# Autodesk Inventor assembly: Shoulder V2
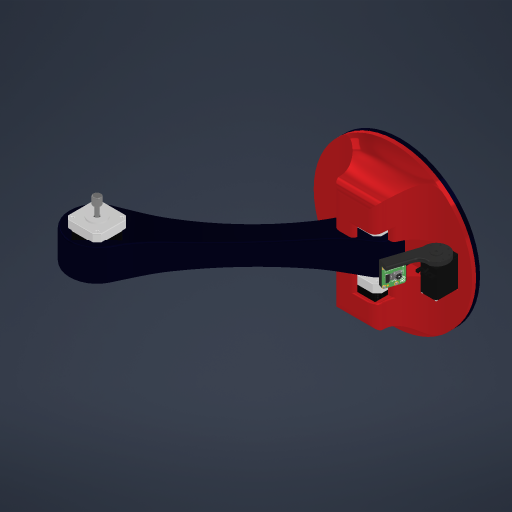
[picture p0: Inventor's stored thumbnail of the model, 512x512]
Saved by Autodesk Inventor 2023 (Build 270158000, 158)
## iProperties
Created: 2023-04-08
Part Number: Shoulder V2
Document SubType Name: Assembly
Designer: vatdu
Author: vatdu
## Documents named in this file (8)
- C:\Users\vatdu\Desktop\CRYSTAL MARK II\Arm\Shoulder\Shoulder V2.iam
- C:\Users\vatdu\Desktop\CRYSTAL MARK II\Components\Stepper Motor.ipt
- C:\Users\vatdu\Desktop\CRYSTAL MARK II\Arm\Shoulder\Rotating Plate.ipt
- C:\Users\vatdu\Desktop\CRYSTAL MARK II\Arm\Shoulder\Motor Cover V2.ipt
- C:\Users\vatdu\Desktop\CRYSTAL MARK II\Arm\Shoulder\Arm.ipt
- C:\Users\vatdu\Desktop\CRYSTAL MARK II\Components\Servo.ipt
- C:\Users\vatdu\Desktop\CRYSTAL MARK II\Components\Camera.iam
- C:\Users\vatdu\Documents\Inventor\Content Center Files\R2023\en-US\BS EN ISO 7045 H\EN ISO 7045 - M1.6 x 3 - 4.8 - H(1).ipt
## Components (13 placed, 7 different names)
1. Stepper Motor:1 — Rigid:3
2. Stepper Motor:2 — Rigid:4, Rigid:6
3. Stepper Motor:3 — Rigid:1, Rotational:2, Rigid:5
4. Rotating Plate:1 — Rotational:1
5. Motor Cover V2:1 — Rigid:1, Rigid:3, Rotational:1
6. Arm:1 — Rigid:4, Rotational:2, Rigid:5, Rigid:6
7. Servo:1 — Rotational:3
8. Camera:1 [sub-assembly] — Rotational:3, Insert:1, Insert:2, Insert:3, Insert:4, Insert:5
9. BS EN ISO 7045 H - Metric M1.6 x 3 - 4.8 - H:1 — Insert:1
10. BS EN ISO 7045 H - Metric M1.6 x 3 - 4.8 - H:2 — Insert:2
11. BS EN ISO 7045 H - Metric M1.6 x 3 - 4.8 - H:3 — Insert:3
12. BS EN ISO 7045 H - Metric M1.6 x 3 - 4.8 - H:4 — Insert:4
13. BS EN ISO 7045 H - Metric M1.6 x 3 - 4.8 - H:5 — Insert:5
## Relationships (13: WeldJoint 5, Insert 5, RevoluteJoint 3)
- Rigid:1 [WeldJoint]: Stepper Motor:3 ↔ Motor Cover V2:1
- Rigid:3 [WeldJoint]: Stepper Motor:1 ↔ Motor Cover V2:1
- Rotational:1 [RevoluteJoint]: Rotating Plate:1 ↔ Motor Cover V2:1
- Rigid:4 [WeldJoint]: Stepper Motor:2 ↔ Arm:1
- Rotational:2 [RevoluteJoint] (-8.05 mm): Stepper Motor:3 ↔ Arm:1
- Rigid:5 [WeldJoint] (-1 mm): Stepper Motor:3 ↔ Arm:1
- Rigid:6 [WeldJoint]: Stepper Motor:2 ↔ Arm:1
- Rotational:3 [RevoluteJoint] (-2.5 mm): Servo:1 ↔ Camera:1
- Insert:1: Camera:1 ↔ BS EN ISO 7045 H - Metric M1.6 x 3 - 4.8 - H:1
- Insert:2: Camera:1 ↔ BS EN ISO 7045 H - Metric M1.6 x 3 - 4.8 - H:2
- Insert:3: Camera:1 ↔ BS EN ISO 7045 H - Metric M1.6 x 3 - 4.8 - H:3
- Insert:4: Camera:1 ↔ BS EN ISO 7045 H - Metric M1.6 x 3 - 4.8 - H:4
- Insert:5: Camera:1 ↔ BS EN ISO 7045 H - Metric M1.6 x 3 - 4.8 - H:5
